# Autodesk Inventor assembly: Assembly
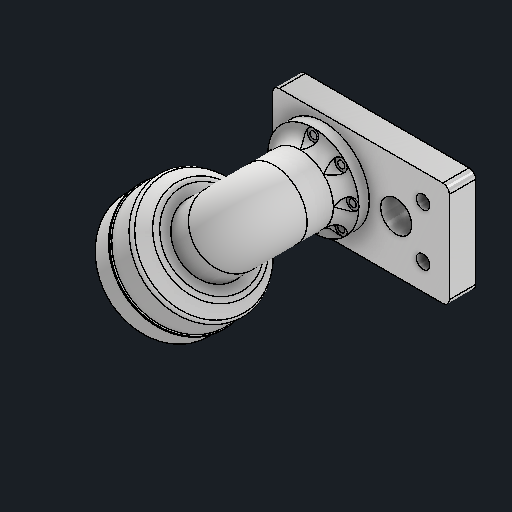
[picture p0: Inventor's stored thumbnail of the model, 512x512]
Saved by Autodesk Inventor 2026.2 (Build 302298000, 298)
## iProperties
Created: 2026-06-17
Part Number: Assembly
Document SubType Name: Assembly
Designer: JoshuaEah
Author: JoshuaEah
## Documents named in this file (6)
- C:\Users\JoshuaEah\Documents\GitHub\Designed-Trinkets\Makera Carvera Air\Air Port\Assembly.iam
- C:\Users\JoshuaEah\Documents\GitHub\Designed-Trinkets\Makera Carvera Air\Air Port\Air Port Plate.ipt
- C:\Users\JoshuaEah\Documents\GitHub\Designed-Trinkets\Makera Carvera Air\Air Port\Outlet.ipt
- C:\Users\JoshuaEah\Documents\GitHub\Designed-Trinkets\Makera Carvera Air\Air Port\Cyclone Hose Adapter.ipt
- C:\Users\JoshuaEah\Documents\GitHub\Designed-Trinkets\Makera Carvera Air\Air Port\Cylone Adapter Sealing Gasket.ipt
- C:\Users\JoshuaEah\Documents\GitHub\Designed-Trinkets\Makera Carvera Air\Air Port\Outlet Gasket.ipt
## Components (5 placed, 5 different names)
1. Air Port Plate:1 — Insert:1, Mate:1, Insert:3
2. Outlet Gasket:1 — Insert:3
3. Outlet:1 — Insert:1, Mate:1, Mate:2, Mate:3
4. Cyclone Hose Adapter:1 — Mate:2, Mate:3, Insert:2
5. Cylone Adapter Sealing Gasket:1 — Insert:2
## Relationships (6: Insert 3, Mate 3)
- Insert:1: Air Port Plate:1 ↔ Outlet:1
- Mate:1: Air Port Plate:1 ↔ Outlet:1
- Mate:2: Outlet:1 ↔ Cyclone Hose Adapter:1
- Mate:3 (-20 mm): Outlet:1 ↔ Cyclone Hose Adapter:1
- Insert:2: Cyclone Hose Adapter:1 ↔ Cylone Adapter Sealing Gasket:1
- Insert:3: Air Port Plate:1 ↔ Outlet Gasket:1
